# Autodesk Inventor assembly: Leg
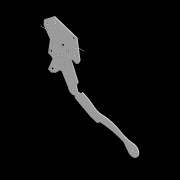
[picture p0: Inventor's stored thumbnail of the model, 180x180]
Saved by Autodesk Inventor 2020 (Build 240168000, 168)
## iProperties
Created: 2020-05-17
Part Number: Leg
Document SubType Name: Assembly
Designer: valer
Author: valer
## Documents named in this file (4)
- C:\Users\valer\Desktop\drummingrobot\src\Leg.iam
- C:\Users\valer\Desktop\drummingrobot\src\Knee.ipt
- C:\Users\valer\Desktop\drummingrobot\src\LowerLeg.ipt
- C:\Users\valer\Desktop\drummingrobot\src\UpperLeg.ipt
## Components (3 placed, 3 different names)
1. Knee:1 — Flush:1, Mate:1, Mate:2, Flush:2, Mate:3
2. LowerLeg:1 — Flush:2, Mate:3
3. UpperLeg:1 — Flush:1, Mate:1, Mate:2
## Relationships (5: Mate 3, Flush 2)
- Flush:1: Knee:1 ↔ UpperLeg:1
- Mate:1: Knee:1 ↔ UpperLeg:1
- Mate:2: Knee:1 ↔ UpperLeg:1
- Flush:2: Knee:1 ↔ LowerLeg:1
- Mate:3: Knee:1 ↔ LowerLeg:1
